# Autodesk Inventor assembly: Tostadora
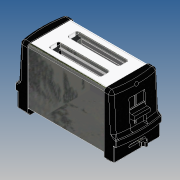
[picture p0: Inventor's stored thumbnail of the model, 180x180]
Saved by Autodesk Inventor 2016 (Build 200138000, 138)
## iProperties
Created: 2016-05-25
Part Number: Tostadora
Document SubType Name: Assembly
Designer: Familia
Author: Familia
## Documents named in this file (8)
- C:\Users\Familia\Desktop\Tostadora\Ensambles\Tostadora.iam
- C:\Users\Familia\Desktop\Tostadora\Partes\Carcaza.ipt
- C:\Users\Familia\Desktop\Tostadora\Partes\Tapa fronta.ipt
- C:\Users\Familia\Desktop\Tostadora\Partes\Tapa lateral.ipt
- C:\Users\Familia\Desktop\Tostadora\Ensambles\Actuador electrico.iam
- C:\Users\Familia\Desktop\Tostadora\Ensambles\Rostizador.iam
- C:\Users\Familia\Desktop\Tostadora\Partes\Tapa del cable.ipt
- C:\Users\Familia\Desktop\Tostadora\Partes\Bandeja recolectora.ipt
## Components (7 placed, 7 different names)
1. Carcaza:1 — Mate:1, Mate:2, Flush:1, Flush:2, Mate:3, Mate:4, Mate:5, Mate:6, Mate:7, Flush:11, Mate:14, Flush:13, Flush:14
2. Tapa fronta:1 — Flush:2, Mate:3, Mate:4, Mate:11, Mate:12
3. Tapa lateral:1 — Mate:5, Mate:6, Mate:7, Mate:15, Mate:16
4. Actuador electrico:1 [sub-assembly] — Flush:11, Mate:11, Mate:12
5. Rostizador:1 [sub-assembly] — Flush:12, Mate:13, Mate:14
6. Tapa del cable:1 — Mate:15, Mate:16
7. Bandeja recolectora:1 — Flush:13, Flush:14
## Relationships (19: Mate 13, Flush 6)
- Mate:1: Carcaza:1
- Mate:2: Carcaza:1
- Flush:1: Carcaza:1
- Flush:2: Carcaza:1 ↔ Tapa fronta:1
- Mate:3: Carcaza:1 ↔ Tapa fronta:1
- Mate:4: Carcaza:1 ↔ Tapa fronta:1
- Mate:5: Carcaza:1 ↔ Tapa lateral:1
- Mate:6: Carcaza:1 ↔ Tapa lateral:1
- Mate:7: Carcaza:1 ↔ Tapa lateral:1
- Flush:11: Carcaza:1 ↔ Actuador electrico:1
- Mate:11 (1 mm): Tapa fronta:1 ↔ Actuador electrico:1
- Mate:12 (7 mm): Tapa fronta:1 ↔ Actuador electrico:1
- Flush:12: Rostizador:1
- Mate:13: Rostizador:1
- Mate:14: Carcaza:1 ↔ Rostizador:1
- Mate:15: Tapa lateral:1 ↔ Tapa del cable:1
- Mate:16: Tapa lateral:1 ↔ Tapa del cable:1
- Flush:13: Carcaza:1 ↔ Bandeja recolectora:1
- Flush:14: Carcaza:1 ↔ Bandeja recolectora:1
